# Autodesk Inventor assembly: GE-12028-04
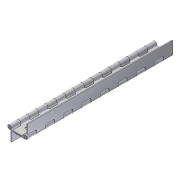
[picture p0: Inventor's stored thumbnail of the model, 180x180]
Saved by Autodesk Inventor 2012 (Build 160160000, 160)
## iProperties
Created: 2008-05-29
Part Number: GE-12028-04
Description: Hinge, Stop Plate
Document SubType Name: Assembly
Designer: dfoster
Author: narosenberg
## Documents named in this file (4)
- C:\Data Folder\FRC 2012 Field\Components\GE-12028-04.iam
- C:\Data Folder\FRC 2012 Field\Components\GE-12028-04A.ipt
- C:\Data Folder\FRC 2012 Field\Components\GE-12028-04B.ipt
- C:\Data Folder\FRC 2012 Field\Components\GE-12028-04C.ipt
## Components (6 placed, 3 different names)
1. GE-12028-04A:1 — Insert:1, Flush:2, Angle:1
2. GE-12028-04A:2 — Flush:1, Mate:1, Insert:2, Angle:2
3. GE-12028-04B:1 — Flush:1, Mate:1, Insert:1, Insert:4, Angle:1
4. GE-12028-04C:1 — Insert:4
5. GE-12028-04A:3 — Flush:2, Insert:2, Insert:3, Angle:2
6. GE-12028-04C:2 — Insert:3
## Relationships (9: Insert 4, Flush 2, Angle 2, Mate 1)
- Flush:1: GE-12028-04A:2 ↔ GE-12028-04B:1
- Mate:1: GE-12028-04A:2 ↔ GE-12028-04B:1
- Insert:1: GE-12028-04A:1 ↔ GE-12028-04B:1
- Insert:4: GE-12028-04B:1 ↔ GE-12028-04C:1
- Flush:2 (-44.45 mm): GE-12028-04A:1 ↔ GE-12028-04A:3
- Insert:2: GE-12028-04A:2 ↔ GE-12028-04A:3
- Insert:3: GE-12028-04A:3 ↔ GE-12028-04C:2
- Angle:1 (-90 deg): GE-12028-04A:1 ↔ GE-12028-04B:1
- Angle:2 (90 deg): GE-12028-04A:2 ↔ GE-12028-04A:3
